# Autodesk Inventor assembly: supportPlate
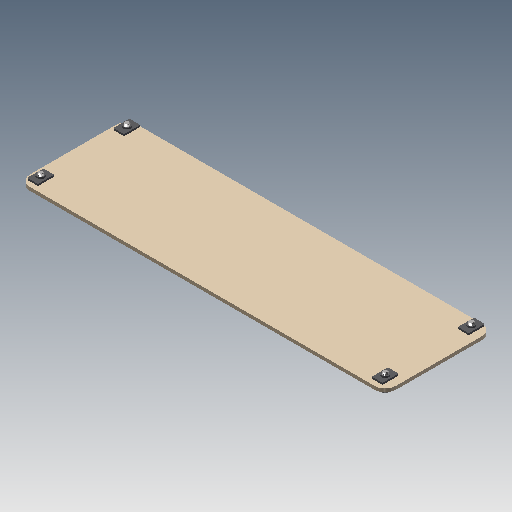
[picture p0: Inventor's stored thumbnail of the model, 512x512]
Saved by Autodesk Inventor 2018 (Build 220112000, 112)
## iProperties
Created: 2017-03-01
Part Number: supportPlate
Document SubType Name: Assembly
Designer: sawaiz
Author: sawaiz
## Documents named in this file (4)
- C:\Users\sawaiz\OneDrive\projects\sPhenixTileTestStand\frame\supportPlate.iam
- C:\Users\sawaiz\OneDrive\projects\sPhenixTileTestStand\frame\supportPlate.ipt
- C:\Users\sawaiz\OneDrive\projects\sPhenixTileTestStand\hardware\m5x10.ipt
- C:\Users\sawaiz\OneDrive\projects\sPhenixTileTestStand\hardware\m5TNut.ipt
## Components (9 placed, 3 different names)
1. supportPlate:1 — Mate:1, Mate:2, Mate:3, Mate:4, Mate:5, Mate:6, Mate:7, Mate:8, Mate:9, Mate:10, Mate:11, Mate:12, Angle:2, Mate:17
2. m5x10:1 — Mate:1, Mate:7, Mate:16
3. m5x10:2 — Mate:2, Mate:8, Mate:15
4. m5x10:3 — Mate:4, Mate:5, Mate:13
5. m5x10:4 — Mate:3, Mate:6, Mate:14
6. m5TNut:1 — Mate:9, Mate:15, Flush:1, Angle:1, Angle:2, Symmetry:1
7. m5TNut:2 — Mate:10, Mate:16, Flush:1
8. m5TNut:3 — Mate:11, Mate:14, Flush:2, Symmetry:2
9. m5TNut:4 — Mate:12, Mate:13, Flush:2, Angle:1, Symmetry:1, Symmetry:2
## Relationships (23: Mate 17, Flush 2, Angle 2, Symmetry 2)
- Mate:1: supportPlate:1 ↔ m5x10:1
- Mate:2: supportPlate:1 ↔ m5x10:2
- Mate:3: supportPlate:1 ↔ m5x10:4
- Mate:4: supportPlate:1 ↔ m5x10:3
- Mate:5: supportPlate:1 ↔ m5x10:3
- Mate:6: supportPlate:1 ↔ m5x10:4
- Mate:7: supportPlate:1 ↔ m5x10:1
- Mate:8: supportPlate:1 ↔ m5x10:2
- Mate:9 (2 mm): supportPlate:1 ↔ m5TNut:1
- Mate:10 (2 mm): supportPlate:1 ↔ m5TNut:2
- Mate:11 (2 mm): supportPlate:1 ↔ m5TNut:3
- Mate:12 (2 mm): supportPlate:1 ↔ m5TNut:4
- Mate:13: m5x10:3 ↔ m5TNut:4
- Mate:14: m5x10:4 ↔ m5TNut:3
- Mate:15: m5x10:2 ↔ m5TNut:1
- Mate:16: m5x10:1 ↔ m5TNut:2
- Flush:1: m5TNut:1 ↔ m5TNut:2
- Flush:2: m5TNut:3 ↔ m5TNut:4
- Angle:1 (0 deg): m5TNut:1 ↔ m5TNut:4
- Angle:2 (0 deg): supportPlate:1 ↔ m5TNut:1
- Symmetry:1: m5TNut:1 ↔ m5TNut:4
- Symmetry:2: m5TNut:3 ↔ m5TNut:4
- Mate:17: supportPlate:1
